# Autodesk Inventor assembly: robot_frame_layer1
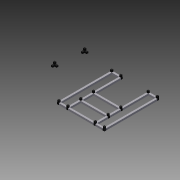
[picture p0: Inventor's stored thumbnail of the model, 180x180]
Saved by Autodesk Inventor 2011 (Build 150239000, 239)
## iProperties
Created: 2013-01-17
Part Number: robot_frame_layer1
Document SubType Name: Assembly
Designer: Christopher
Author: Christopher
## Documents named in this file (10)
- F:\Users\Christopher\Documents\GitHub\2013CAD\2013 robot\forklift\robot parts\robot_frame_layer1.iam
- F:\Users\Christopher\Documents\GitHub\2013CAD\2013 robot\forklift\robot parts\1tube_4_layer1_outside.ipt
- F:\Users\Christopher\Documents\GitHub\2013CAD\2013 robot\forklift\robot parts\1tube_6_layer1_boardsupportsupport.ipt
- F:\Users\Christopher\Documents\GitHub\2013CAD\2013 robot\forklift\robot parts\1tube_6_layer1_motorsupport.ipt
- F:\Users\Christopher\Documents\GitHub\2013CAD\2013 robot\forklift\robot parts\1tube_14_layer1_innersupport.ipt
- F:\Users\Christopher\Documents\GitHub\2013CAD\2013 robot\forklift\robot parts\1tube_14_layer1_inside.ipt
- F:\Users\Christopher\Documents\GitHub\2013CAD\2013 robot\forklift\robot parts\1tube_14_layer1_outside.ipt
- F:\Users\Christopher\Documents\GitHub\2013CAD\2013 robot\forklift\robot parts\1tube_28_layer1_outside.ipt
- F:\Users\Christopher\Documents\GitHub\2013CAD\2013 robot\forklift\Misc parts\3-way corner.ipt
- F:\Users\Christopher\Documents\GitHub\2013CAD\2013 robot\forklift\Misc parts\4-way corner.ipt
## Components (29 placed, 9 different names)
1. 1tube_4_layer1_outside:1 — Mate:7, Mate:8, Mate:9, Mate:10, Mate:11, Mate:12
2. 1tube_6_layer1_boardsupportsupport:1 — Mate:22, Mate:23, Mate:24, Mate:25, Mate:26, Mate:27
3. 1tube_6_layer1_motorsupport:1 — Mate:28, Mate:29, Mate:30, Mate:34, Mate:35, Mate:36
4. 1tube_14_layer1_innersupport:1 — Mate:31, Mate:32, Mate:33, Mate:46, Mate:47, Mate:48
5. 1tube_14_layer1_inside:1 — Mate:37, Mate:38, Mate:39
6. 1tube_14_layer1_outside:1 — Mate:19, Mate:20, Mate:21, Mate:49, Mate:50, Mate:51
7. 1tube_28_layer1_outside:1 — Mate:1, Mate:2, Mate:3, Mate:4, Mate:5, Mate:6
8. 3-way corner:1 — Mate:1, Mate:2, Mate:3, Mate:13, Mate:14, Mate:15
9. 4-way corner:1 — Mate:43, Mate:44, Mate:45, Mate:55, Mate:56, Mate:57, Mate:58, Mate:59, Mate:60
10. 3-way corner:2 — Mate:4, Mate:5, Mate:6, Mate:7, Mate:8, Mate:9
11. 3-way corner:3
12. 3-way corner:4 — Mate:61, Mate:62, Mate:63, Mate:70, Mate:71, Mate:72
13. 3-way corner:5 — Mate:73, Mate:74, Mate:75, Mate:77
14. 3-way corner:6 — Mate:67, Mate:68, Mate:69, Mate:76, Mate:78
15. 3-way corner:7 — Mate:16, Mate:17, Mate:18, Mate:37, Mate:38, Mate:39
16. 3-way corner:8
17. 4-way corner:2 — Mate:10, Mate:11, Mate:12, Mate:19, Mate:20, Mate:21, Mate:22, Mate:23, Mate:24
18. 1tube_4_layer1_outside:2 — Mate:13, Mate:14, Mate:15, Mate:16, Mate:17, Mate:18
19. 4-way corner:3 — Mate:25, Mate:26, Mate:27, Mate:28, Mate:29, Mate:30, Mate:31, Mate:32, Mate:33
20. 4-way corner:4 — Mate:34, Mate:35, Mate:36, Mate:40, Mate:41, Mate:42
21. 1tube_14_layer1_innersupport:2 — Mate:40, Mate:41, Mate:42, Mate:43, Mate:44, Mate:45
22. 4-way corner:5 — Mate:46, Mate:47, Mate:48, Mate:53, Mate:54
23. 4-way corner:6 — Mate:49, Mate:50, Mate:51, Mate:52, Mate:64, Mate:65, Mate:66
24. 1tube_6_layer1_motorsupport:2 — Mate:55, Mate:56, Mate:57
25. 1tube_6_layer1_boardsupportsupport:2 — Mate:52, Mate:53, Mate:54
26. 1tube_14_layer1_inside:2 — Mate:58, Mate:59, Mate:60, Mate:61, Mate:62, Mate:63
27. 1tube_4_layer1_outside:3 — Mate:64, Mate:65, Mate:66, Mate:67, Mate:68, Mate:69
28. 1tube_4_layer1_outside:4 — Mate:70, Mate:71, Mate:72, Mate:73, Mate:74, Mate:75
29. 1tube_28_layer1_outside:2 — Mate:76, Mate:77, Mate:78
## Relationships (78: Mate 78)
- Mate:1: 1tube_28_layer1_outside:1 ↔ 3-way corner:1
- Mate:2: 1tube_28_layer1_outside:1 ↔ 3-way corner:1
- Mate:3: 1tube_28_layer1_outside:1 ↔ 3-way corner:1
- Mate:4: 1tube_28_layer1_outside:1 ↔ 3-way corner:2
- Mate:5: 1tube_28_layer1_outside:1 ↔ 3-way corner:2
- Mate:6: 1tube_28_layer1_outside:1 ↔ 3-way corner:2
- Mate:7: 1tube_4_layer1_outside:1 ↔ 3-way corner:2
- Mate:8: 1tube_4_layer1_outside:1 ↔ 3-way corner:2
- Mate:9: 1tube_4_layer1_outside:1 ↔ 3-way corner:2
- Mate:10: 1tube_4_layer1_outside:1 ↔ 4-way corner:2
- Mate:11: 1tube_4_layer1_outside:1 ↔ 4-way corner:2
- Mate:12: 1tube_4_layer1_outside:1 ↔ 4-way corner:2
- Mate:13: 3-way corner:1 ↔ 1tube_4_layer1_outside:2
- Mate:14: 3-way corner:1 ↔ 1tube_4_layer1_outside:2
- Mate:15: 3-way corner:1 ↔ 1tube_4_layer1_outside:2
- Mate:16: 3-way corner:7 ↔ 1tube_4_layer1_outside:2
- Mate:17: 3-way corner:7 ↔ 1tube_4_layer1_outside:2
- Mate:18: 3-way corner:7 ↔ 1tube_4_layer1_outside:2
- Mate:19: 1tube_14_layer1_outside:1 ↔ 4-way corner:2
- Mate:20: 1tube_14_layer1_outside:1 ↔ 4-way corner:2
- Mate:21: 1tube_14_layer1_outside:1 ↔ 4-way corner:2
- Mate:22: 1tube_6_layer1_boardsupportsupport:1 ↔ 4-way corner:2
- Mate:23: 1tube_6_layer1_boardsupportsupport:1 ↔ 4-way corner:2
- Mate:24: 1tube_6_layer1_boardsupportsupport:1 ↔ 4-way corner:2
- Mate:25: 1tube_6_layer1_boardsupportsupport:1 ↔ 4-way corner:3
- Mate:26: 1tube_6_layer1_boardsupportsupport:1 ↔ 4-way corner:3
- Mate:27: 1tube_6_layer1_boardsupportsupport:1 ↔ 4-way corner:3
- Mate:28: 1tube_6_layer1_motorsupport:1 ↔ 4-way corner:3
- Mate:29: 1tube_6_layer1_motorsupport:1 ↔ 4-way corner:3
- Mate:30: 1tube_6_layer1_motorsupport:1 ↔ 4-way corner:3
- Mate:31: 1tube_14_layer1_innersupport:1 ↔ 4-way corner:3
- Mate:32: 1tube_14_layer1_innersupport:1 ↔ 4-way corner:3
- Mate:33: 1tube_14_layer1_innersupport:1 ↔ 4-way corner:3
- Mate:34: 1tube_6_layer1_motorsupport:1 ↔ 4-way corner:4
- Mate:35: 1tube_6_layer1_motorsupport:1 ↔ 4-way corner:4
- Mate:36: 1tube_6_layer1_motorsupport:1 ↔ 4-way corner:4
- Mate:37: 1tube_14_layer1_inside:1 ↔ 3-way corner:7
- Mate:38: 1tube_14_layer1_inside:1 ↔ 3-way corner:7
- Mate:39: 1tube_14_layer1_inside:1 ↔ 3-way corner:7
- Mate:40: 4-way corner:4 ↔ 1tube_14_layer1_innersupport:2
- Mate:41: 4-way corner:4 ↔ 1tube_14_layer1_innersupport:2
- Mate:42: 4-way corner:4 ↔ 1tube_14_layer1_innersupport:2
- Mate:43: 4-way corner:1 ↔ 1tube_14_layer1_innersupport:2
- Mate:44: 4-way corner:1 ↔ 1tube_14_layer1_innersupport:2
- Mate:45: 4-way corner:1 ↔ 1tube_14_layer1_innersupport:2
- Mate:46: 1tube_14_layer1_innersupport:1 ↔ 4-way corner:5
- Mate:47: 1tube_14_layer1_innersupport:1 ↔ 4-way corner:5
- Mate:48: 1tube_14_layer1_innersupport:1 ↔ 4-way corner:5
- Mate:49: 1tube_14_layer1_outside:1 ↔ 4-way corner:6
- Mate:50: 1tube_14_layer1_outside:1 ↔ 4-way corner:6
- Mate:51: 1tube_14_layer1_outside:1 ↔ 4-way corner:6
- Mate:52: 4-way corner:6 ↔ 1tube_6_layer1_boardsupportsupport:2
- Mate:53: 4-way corner:5 ↔ 1tube_6_layer1_boardsupportsupport:2
- Mate:54: 4-way corner:5 ↔ 1tube_6_layer1_boardsupportsupport:2
- Mate:55: 4-way corner:1 ↔ 1tube_6_layer1_motorsupport:2
- Mate:56: 4-way corner:1 ↔ 1tube_6_layer1_motorsupport:2
- Mate:57: 4-way corner:1 ↔ 1tube_6_layer1_motorsupport:2
- Mate:58: 4-way corner:1 ↔ 1tube_14_layer1_inside:2
- Mate:59: 4-way corner:1 ↔ 1tube_14_layer1_inside:2
- Mate:60: 4-way corner:1 ↔ 1tube_14_layer1_inside:2
- Mate:61: 3-way corner:4 ↔ 1tube_14_layer1_inside:2
- Mate:62: 3-way corner:4 ↔ 1tube_14_layer1_inside:2
- Mate:63: 3-way corner:4 ↔ 1tube_14_layer1_inside:2
- Mate:64: 4-way corner:6 ↔ 1tube_4_layer1_outside:3
- Mate:65: 4-way corner:6 ↔ 1tube_4_layer1_outside:3
- Mate:66: 4-way corner:6 ↔ 1tube_4_layer1_outside:3
- Mate:67: 3-way corner:6 ↔ 1tube_4_layer1_outside:3
- Mate:68: 3-way corner:6 ↔ 1tube_4_layer1_outside:3
- Mate:69: 3-way corner:6 ↔ 1tube_4_layer1_outside:3
- Mate:70: 3-way corner:4 ↔ 1tube_4_layer1_outside:4
- Mate:71: 3-way corner:4 ↔ 1tube_4_layer1_outside:4
- Mate:72: 3-way corner:4 ↔ 1tube_4_layer1_outside:4
- Mate:73: 3-way corner:5 ↔ 1tube_4_layer1_outside:4
- Mate:74: 3-way corner:5 ↔ 1tube_4_layer1_outside:4
- Mate:75: 3-way corner:5 ↔ 1tube_4_layer1_outside:4
- Mate:76: 3-way corner:6 ↔ 1tube_28_layer1_outside:2
- Mate:77: 3-way corner:5 ↔ 1tube_28_layer1_outside:2
- Mate:78: 3-way corner:6 ↔ 1tube_28_layer1_outside:2
